# Autodesk Inventor assembly: писюны
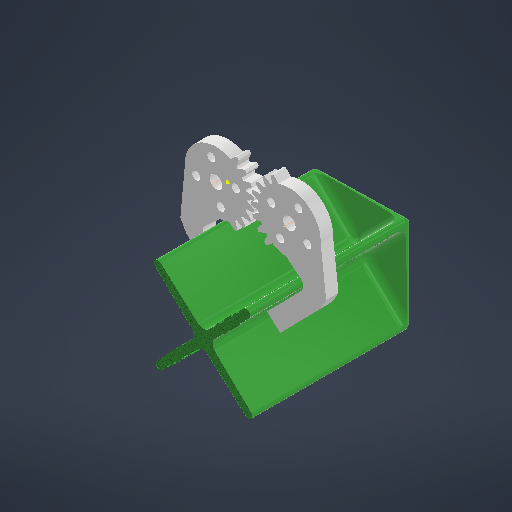
[picture p0: Inventor's stored thumbnail of the model, 512x512]
Saved by Autodesk Inventor 2025 (Build 290162000, 162)
## iProperties
Created: 2024-12-28
Part Number: писюны
Document SubType Name: Assembly
Designer: Phantom
Author: Phantom
## Documents named in this file (5)
- C:\Users\GameHD\Desktop\phantom 16950\писюны.iam
- C:\Users\GameHD\Desktop\phantom 16950\am-5401 Sample.ipt
- C:\Users\GameHD\Desktop\phantom 16950\писюн.ipt
- C:\Users\GameHD\Desktop\phantom 16950\писюн 2.ipt
- C:\Users\GameHD\Downloads\Telegram Desktop\Клешни с фиксатором\Клешни с фиксатором.ipt
## Components (4 placed, 4 different names)
1. am-5401 Sample:1 — Заподлицо:1, Заподлицо:2
2. Клешни с фиксатором:4
3. писюн 2:1 — Заподлицо:2, Совмещение:2, Совмещение:5
4. писюн:1 — Заподлицо:1, Совмещение:3, Совмещение:4
## Relationships (6: Mate 4, Flush 2)
- Заподлицо:1 [Flush] (-40 mm): am-5401 Sample:1 ↔ писюн:1
- Заподлицо:2 [Flush] (-40 mm): am-5401 Sample:1 ↔ писюн 2:1
- Совмещение:2 [Mate]: писюн 2:1
- Совмещение:3 [Mate]: писюн:1
- Совмещение:4 [Mate]: писюн:1
- Совмещение:5 [Mate]: писюн 2:1
